# Autodesk Inventor assembly: Right side collector assembly_MIR1_MIR
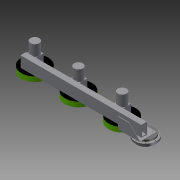
[picture p0: Inventor's stored thumbnail of the model, 180x180]
Saved by Autodesk Inventor 2015 (Build 190159000, 159)
## iProperties
Created: 2015-01-20
Part Number: Right side collector assembly_MIR1_MIR
Document SubType Name: Assembly
Designer: szymsea16
Author: chapale16
## Documents named in this file (3)
- \\lhssvr02\Homedirs\Robotics Club\CAD Model 2015\CDR prep\Tote Collector Arms\Right side collector assembly_MIR1_MIR.iam
- \\lhssvr02\Homedirs\Robotics Club\CAD Model 2015\Igus and Arm Bracket_MIR4_MIR.iam
- \\lhssvr02\Homedirs\Robotics Club\CAD Model 2015\CDR prep\Tote Collector Arms\Collector Arms v2.0_MIR_MIR_MIR2_MIR.iam
## Components (2 placed, 2 different names)
1. Igus and Arm Bracket_MIR4_MIR:1 [sub-assembly] — Flush:1, Mate:3, Mate:2, Mate:1
2. Collector Arms v2.0_MIR_MIR_MIR2_MIR:1 [sub-assembly] — Flush:1, Mate:3, Mate:2, Mate:1
## Relationships (4: Mate 3, Flush 1)
- Flush:1: Igus and Arm Bracket_MIR4_MIR:1 ↔ Collector Arms v2.0_MIR_MIR_MIR2_MIR:1
- Mate:3: Igus and Arm Bracket_MIR4_MIR:1 ↔ Collector Arms v2.0_MIR_MIR_MIR2_MIR:1
- Mate:2: Igus and Arm Bracket_MIR4_MIR:1 ↔ Collector Arms v2.0_MIR_MIR_MIR2_MIR:1
- Mate:1: Igus and Arm Bracket_MIR4_MIR:1 ↔ Collector Arms v2.0_MIR_MIR_MIR2_MIR:1
